# Autodesk Inventor assembly: Assembly1
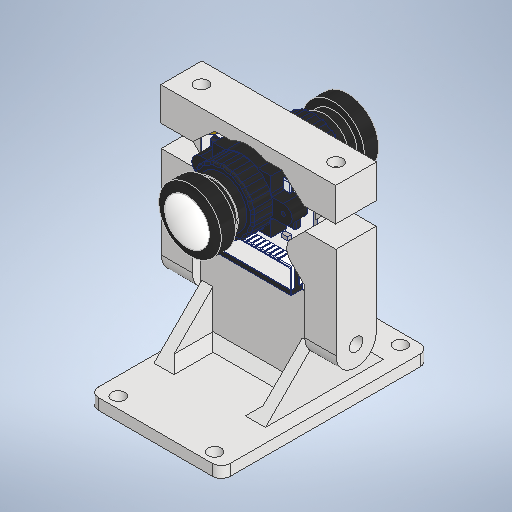
[picture p0: Inventor's stored thumbnail of the model, 512x512]
Saved by Autodesk Inventor 2025.1 (Build 291241000, 241)
## iProperties
Created: 2026-04-04
Part Number: Assembly1
Document SubType Name: Assembly
Designer: User
Author: User
## Documents named in this file (8)
- D:\One Drive\OneDrive - Politeknik Sultan Salahuddin Abdul Aziz Shah\Documents\Inventor\RobosotPSA\Assembly1.iam
- D:\One Drive\OneDrive - Politeknik Sultan Salahuddin Abdul Aziz Shah\Documents\Inventor\RobosotPSA\rpiCameraMAssembly\rpiCameraMAssembly\rpiCameraMAssembly.ipt
- D:\One Drive\OneDrive - Politeknik Sultan Salahuddin Abdul Aziz Shah\Documents\Inventor\RobosotPSA\cameraholder.ipt
- D:\One Drive\OneDrive - Politeknik Sultan Salahuddin Abdul Aziz Shah\Documents\Inventor\RobosotPSA\Kamera_Schraube_Tripod\Kamera_Schraube_Tripod\Kamera_Schraube_Tripod.ipt
- D:\One Drive\OneDrive - Politeknik Sultan Salahuddin Abdul Aziz Shah\Documents\Inventor\RobosotPSA\FOVcam.ipt
- D:\One Drive\OneDrive - Politeknik Sultan Salahuddin Abdul Aziz Shah\Documents\Inventor\RobosotPSA\cameraholder_v2.ipt
- D:\One Drive\OneDrive - Politeknik Sultan Salahuddin Abdul Aziz Shah\Documents\Inventor\RobosotPSA\CameraTopSlider.ipt
- D:\One Drive\OneDrive - Politeknik Sultan Salahuddin Abdul Aziz Shah\Documents\Inventor\RobosotPSA\SideCameraSlider.ipt
## Components (10 placed, 7 different names)
1. cameraholder:1 — Mate:1, Mate:2, Mate:3, Mate:4, Mate:5, Mate:6, Mate:7, Mate:8
2. Kamera_Schraube_Tripod:1 — Mate:1
3. rpiCameraMAssembly:2 — Mate:2, Mate:3, Mate:4, Mate:5, Mate:9, Mate:10
4. rpiCameraMAssembly:3 — Mate:6, Mate:7, Mate:8, Flush:4, Flush:5
5. FOVcam:1 — Flush:1, Flush:2
6. FOVcam:2 — Flush:1, Flush:2
7. cameraholder_v2:1 — Mate:9, Flush:3, Mate:11
8. CameraTopSlider:1 — Flush:3
9. SideCameraSlider:1 — Flush:4, Flush:5, Mate:12
10. SideCameraSlider:2 — Mate:10, Mate:11, Mate:12
## Relationships (17: Mate 12, Flush 5)
- Mate:1: cameraholder:1 ↔ Kamera_Schraube_Tripod:1
- Mate:2: cameraholder:1 ↔ rpiCameraMAssembly:2
- Mate:3: cameraholder:1 ↔ rpiCameraMAssembly:2
- Mate:4: cameraholder:1 ↔ rpiCameraMAssembly:2
- Mate:5: cameraholder:1 ↔ rpiCameraMAssembly:2
- Mate:6: cameraholder:1 ↔ rpiCameraMAssembly:3
- Mate:7: cameraholder:1 ↔ rpiCameraMAssembly:3
- Mate:8: cameraholder:1 ↔ rpiCameraMAssembly:3
- Flush:1: FOVcam:1 ↔ FOVcam:2
- Flush:2: FOVcam:1 ↔ FOVcam:2
- Mate:9: rpiCameraMAssembly:2 ↔ cameraholder_v2:1
- Flush:3: cameraholder_v2:1 ↔ CameraTopSlider:1
- Flush:4: rpiCameraMAssembly:3 ↔ SideCameraSlider:1
- Flush:5: rpiCameraMAssembly:3 ↔ SideCameraSlider:1
- Mate:10: rpiCameraMAssembly:2 ↔ SideCameraSlider:2
- Mate:11: cameraholder_v2:1 ↔ SideCameraSlider:2
- Mate:12: SideCameraSlider:1 ↔ SideCameraSlider:2
